# Autodesk Inventor assembly: RC5
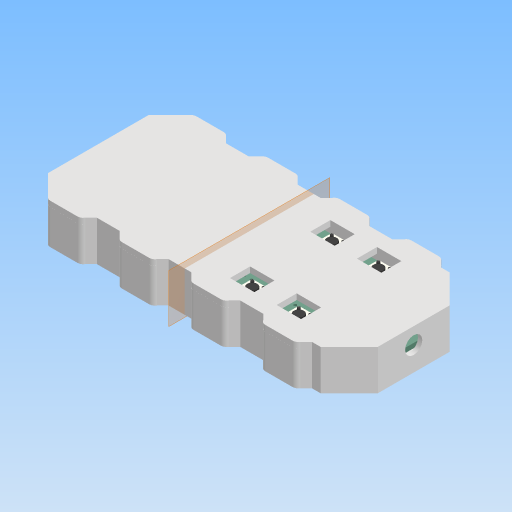
[picture p0: Inventor's stored thumbnail of the model, 512x512]
Saved by Autodesk Inventor 2024 (Build 280153000, 153)
## iProperties
Created: 2024-03-14
Part Number: RC5
Document SubType Name: Assembly
Designer: MenMe
Author: MenMe
## Documents named in this file (4)
- C:\Users\MenMe\Documents\GitHub\RoboCop\- 3D -\other\RC5.iam
- C:\Users\MenMe\Documents\GitHub\RoboCop\- 3D -\other\RC5 Controller.ipt
- C:\Users\MenMe\Documents\GitHub\RoboCop\- 3D -\other\RC5 Controller kryt.ipt
- C:\Users\MenMe\Documents\GitHub\RoboCop\- PCB -\RC-5 Remote Controler\RC-5 Remote Controler\RC-5 Remote Controler.iam
## Components (3 placed, 3 different names)
1. RC5 Controller:1 — Mate:1, Mate:2, Mate:3, Mate:4, Mate:5
2. RC5 Controller kryt:1 — Mate:3, Mate:4, Mate:5
3. RC-5 Remote Controler:1 [sub-assembly] — Mate:1, Mate:2
## Relationships (5: Mate 5)
- Mate:1: RC5 Controller:1 ↔ RC-5 Remote Controler:1
- Mate:2: RC5 Controller:1 ↔ RC-5 Remote Controler:1
- Mate:3: RC5 Controller:1 ↔ RC5 Controller kryt:1
- Mate:4: RC5 Controller:1 ↔ RC5 Controller kryt:1
- Mate:5: RC5 Controller:1 ↔ RC5 Controller kryt:1
